# Autodesk Inventor assembly: Main
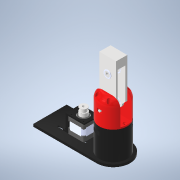
[picture p0: Inventor's stored thumbnail of the model, 180x180]
Saved by Autodesk Inventor 2022.3 (Build 263350000, 350)
## iProperties
Created: 2022-05-27
Part Number: Main
Document SubType Name: Assembly
Designer: Mlees
Author: Mlees
## Documents named in this file (13)
- D:\504Engineering\Project_0000\Designs\Design_5\Main.iam
- D:\504Engineering\Project_0000\Designs\Design_5\Downloaded_Parts\127076899-9-stp-mtrl-14034_nema_14\stp-mtrl-14034.ipt
- D:\504Engineering\Project_0000\Designs\Design_5\Created_Parts\GT2 20T.ipt
- D:\504Engineering\Project_0000\Designs\Design_5\Created_Parts\Base.ipt
- D:\504Engineering\Project_0000\Designs\Design_5\Created_Parts\Motor_Mount.ipt
- D:\504Engineering\Project_0000\Designs\Design_5\Created_Parts\GT2 60T.ipt
- D:\504Engineering\Project_0000\Designs\Design_5\Downloaded_Parts\4668K334_Permanently Lubricated Stainless Steel Ball Bearing 688-2RS.ipt
- D:\504Engineering\Project_0000\Designs\Design_5\Downloaded_Parts\4634T11_Multipurpose 6061 Aluminum 5mm rod.ipt
- D:\504Engineering\Project_0000\Designs\Design_5\Created_Parts\Base_To_First_Tilt_Attachment.ipt
- D:\504Engineering\Project_0000\Designs\Design_5\Created_Parts\tilt_1_base.ipt
- D:\504Engineering\Project_0000\Designs\Design_5\Downloaded_Parts\4634T11_Multipurpose 6061 Aluminum 5mm rod_Tilt_Shaft.ipt
- D:\504Engineering\Project_0000\Designs\Design_5\Downloaded_Parts\6153K15_Stainless Steel Ball Bearing.ipt
- D:\504Engineering\Project_0000\Designs\Design_5\Created_Parts\Joint1.ipt
## Components (15 placed, 12 different names)
1. stp-mtrl-14034:1 — Mate:1, Mate:2, Mate:6, Mate:7
2. GT2 20T:1 — Mate:1, Mate:2
3. Base:1 — Mate:5, Mate:8, Mate:9, Mate:14, Mate:15, Mate:34
4. Motor_Mount:1 — Mate:5, Mate:6, Mate:7, Mate:34
5. GT2 60T:1 — Mate:8, Mate:9, Mate:18, Flush:1, Mate:19, Mate:20
6. 4668K334_Permanently Lubricated Stainless Steel Ball Bearing 688-2RS:2 — Mate:14, Mate:15
7. 4634T11_Multipurpose 6061 Aluminum 5mm rod:1 — Mate:18, Flush:1
8. Base_To_First_Tilt_Attachment:1 — Mate:19, Mate:20, Mate:23, Mate:24, Mate:25
9. tilt_1_base:1 — Mate:23, Mate:24, Mate:25, Mate:27, Mate:28, Mate:29, Mate:33
10. GT2 20T:2 — Mate:26, Mate:29
11. 4634T11_Multipurpose 6061 Aluminum 5mm rod_Tilt_Shaft:1 — Mate:26, Mate:27, Mate:28, Mate:32
12. 6153K15_Stainless Steel Ball Bearing:2 — Mate:31, Flush:3, Mate:32
13. Joint1:1 — Mate:31, Flush:3, Mate:33, Mate:35, Mate:36, Flush:4, Flush:5
14. 6153K15_Stainless Steel Ball Bearing:3 — Mate:35, Flush:5
15. 6153K15_Stainless Steel Ball Bearing:4 — Mate:36, Flush:4
## Relationships (29: Mate 25, Flush 4)
- Mate:1: stp-mtrl-14034:1 ↔ GT2 20T:1
- Mate:2 (1 mm): stp-mtrl-14034:1 ↔ GT2 20T:1
- Mate:5: Base:1 ↔ Motor_Mount:1
- Mate:6: stp-mtrl-14034:1 ↔ Motor_Mount:1
- Mate:7: stp-mtrl-14034:1 ↔ Motor_Mount:1
- Mate:8: Base:1 ↔ GT2 60T:1
- Mate:9: Base:1 ↔ GT2 60T:1
- Mate:14: Base:1 ↔ 4668K334_Permanently Lubricated Stainless Steel Ball Bearing 688-2RS:2
- Mate:15: Base:1 ↔ 4668K334_Permanently Lubricated Stainless Steel Ball Bearing 688-2RS:2
- Mate:18: GT2 60T:1 ↔ 4634T11_Multipurpose 6061 Aluminum 5mm rod:1
- Flush:1: GT2 60T:1 ↔ 4634T11_Multipurpose 6061 Aluminum 5mm rod:1
- Mate:19: GT2 60T:1 ↔ Base_To_First_Tilt_Attachment:1
- Mate:20: GT2 60T:1 ↔ Base_To_First_Tilt_Attachment:1
- Mate:23: Base_To_First_Tilt_Attachment:1 ↔ tilt_1_base:1
- Mate:24: Base_To_First_Tilt_Attachment:1 ↔ tilt_1_base:1
- Mate:25: Base_To_First_Tilt_Attachment:1 ↔ tilt_1_base:1
- Mate:26: GT2 20T:2 ↔ 4634T11_Multipurpose 6061 Aluminum 5mm rod_Tilt_Shaft:1
- Mate:27: tilt_1_base:1 ↔ 4634T11_Multipurpose 6061 Aluminum 5mm rod_Tilt_Shaft:1
- Mate:28 (-5 mm): tilt_1_base:1 ↔ 4634T11_Multipurpose 6061 Aluminum 5mm rod_Tilt_Shaft:1
- Mate:29 (7 mm): tilt_1_base:1 ↔ GT2 20T:2
- Mate:31: 6153K15_Stainless Steel Ball Bearing:2 ↔ Joint1:1
- Flush:3: 6153K15_Stainless Steel Ball Bearing:2 ↔ Joint1:1
- Mate:32: 4634T11_Multipurpose 6061 Aluminum 5mm rod_Tilt_Shaft:1 ↔ 6153K15_Stainless Steel Ball Bearing:2
- Mate:33: tilt_1_base:1 ↔ Joint1:1
- Mate:34 (-4.5 mm): Base:1 ↔ Motor_Mount:1
- Mate:35: Joint1:1 ↔ 6153K15_Stainless Steel Ball Bearing:3
- Mate:36: Joint1:1 ↔ 6153K15_Stainless Steel Ball Bearing:4
- Flush:4: Joint1:1 ↔ 6153K15_Stainless Steel Ball Bearing:4
- Flush:5: Joint1:1 ↔ 6153K15_Stainless Steel Ball Bearing:3
